# Autodesk Inventor assembly: 大粗轴四方轴套
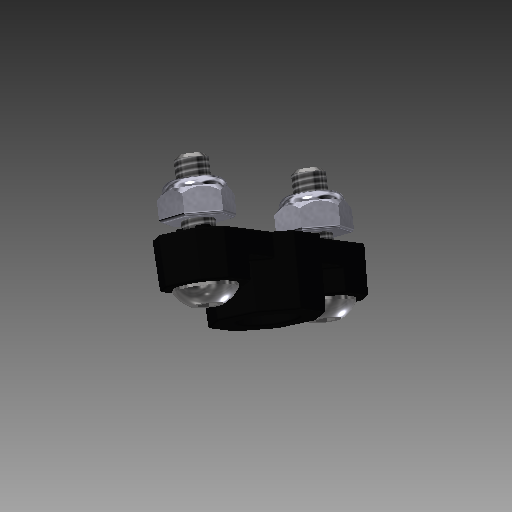
[picture p0: Inventor's stored thumbnail of the model, 512x512]
Saved by Autodesk Inventor 2019.3 (Build 233278000, 278)
## iProperties
Created: 2019-03-29
Part Number: 大粗轴四方轴套
Material: 常规
Document SubType Name: Assembly
Designer: 10731
Mass: 22.5002 g
Surface Area: 29.8355 cm^2
Volume: 2.87965 cm^3
Density: 7.8135 g/cm^3
Author: 10731
## Documents named in this file (4)
- D:\cad\零件库\大粗轴四方轴套.iam
- D:\cad\零件库\垫片轴套大白等\Bearing Block HS.ipt
- D:\cad\零件库\螺丝螺帽\Screw 8-32 x 0.625'' - Black.ipt
- D:\cad\零件库\螺丝螺帽\Nut 8-32 Nylock.ipt
## Components (5 placed, 3 different names)
1. Bearing Block HS:1
2. Screw 8-32 x 0.625'' - Black:1
3. Screw 8-32 x 0.625'' - Black:2
4. Nut 8-32 Nylock:1
5. Nut 8-32 Nylock:2
## Relationships (8: Mate 8)
- [Mate]: Bearing Block HS:1 ↔ Screw 8-32 x 0.625'' - Black:1
- [Mate]: Bearing Block HS:1 ↔ Screw 8-32 x 0.625'' - Black:2
- [Mate]: Bearing Block HS:1 ↔ Screw 8-32 x 0.625'' - Black:1
- [Mate]: Bearing Block HS:1 ↔ Screw 8-32 x 0.625'' - Black:2
- [Mate]: Screw 8-32 x 0.625'' - Black:1 ↔ Nut 8-32 Nylock:1
- [Mate] (1.6 mm): Bearing Block HS:1 ↔ Nut 8-32 Nylock:1
- [Mate]: Screw 8-32 x 0.625'' - Black:2 ↔ Nut 8-32 Nylock:2
- [Mate] (1.6 mm): Bearing Block HS:1 ↔ Nut 8-32 Nylock:2
